# Autodesk Inventor assembly: WCP-0075
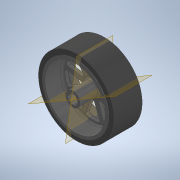
[picture p0: Inventor's stored thumbnail of the model, 180x180]
Saved by Autodesk Inventor 2020 (Build 240168000, 168)
## iProperties
Created: 2022-01-10
Part Number: WCP-0075
Document SubType Name: Assembly
Designer: 23kaltomare
Author: 23kaltomare
## Documents named in this file (3)
- T:\EIT\2022 Rapid React\COMMON PARTS\WHEELS\WCP-0075.iam
- T:\EIT\2022 Rapid React\COMMON PARTS\WHEELS\WCP-0075.ipt
- T:\EIT\2022 Rapid React\COMMON PARTS\WHEELS\WCP-0075-tread.ipt
## Components (2 placed, 2 different names)
1. WCP-0075:1 — Insert:1
2. WCP-0075-tread:1 — Insert:1
## Relationships (1: Insert 1)
- Insert:1: WCP-0075:1 ↔ WCP-0075-tread:1
